# Autodesk Inventor assembly: 拨盘体
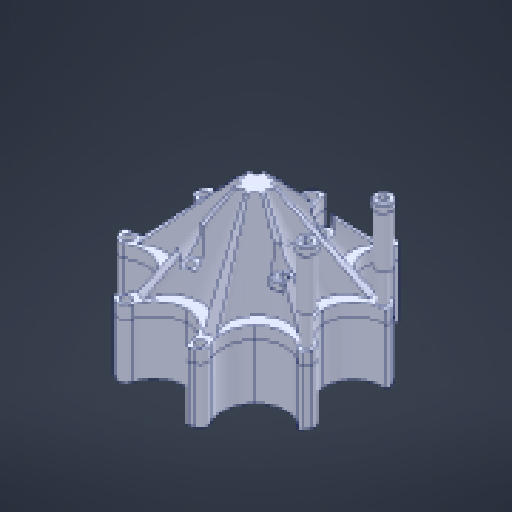
[picture p0: Inventor's stored thumbnail of the model, 512x512]
Saved by Autodesk Inventor 2025 (Build 290162000, 162)
## iProperties
Created: 2025-12-23
Part Number: 拨盘体
Document SubType Name: Assembly
Designer: XH
Author: XH
Revision Number: ä»
## Documents named in this file (8)
- C:\1A_Engineering_files\RCInventor\铝件版本\拨弹盘\拨盘体.iam
- C:\1A_Engineering_files\RCInventor\铝件版本\拨弹盘\八爪拨盘柱体.ipt
- C:\1A_Engineering_files\RCInventor\铝件版本\拨弹盘\八爪拨盘平面盘体.ipt
- C:\1A_Engineering_files\RCInventor\铝件版本\拨弹盘\2X铜嵌件M3-外5-长8.ipt
- C:\1A_Engineering_files\RCInventor\铝件版本\拨弹盘\螺栓M3-30.ipt
- C:\1A_Engineering_files\RCInventor\铝件版本\拨弹盘\斜坡滑槽.ipt
- C:\1A_Engineering_files\RCInventor\铝件版本\拨弹盘\螺栓M3-10.ipt
- C:\1A_Engineering_files\RCInventor\铝件版本\拨弹盘\螺栓M3-12.ipt
## Components (10 placed, 10 different names)
1. 八爪拨盘柱体_11 — 配合:1, 配合:2, 配合:3
2. 八爪拨盘平面盘体_12 — 配合:1, 配合:2, 配合:3
3. 螺栓M3-30_18
4. 螺栓M3-30_19
5. 2X铜嵌件M3-外5-长8_25
6. 2X铜嵌件M3-外5-长8_26
7. 斜坡滑槽_29
8. 螺栓M3-10_31
9. 螺栓M3-12_34
10. 螺栓M3-12_35
## Relationships (3: Mate 3)
- 配合:1 [Mate]: 八爪拨盘柱体_11 ↔ 八爪拨盘平面盘体_12
- 配合:2 [Mate]: 八爪拨盘柱体_11 ↔ 八爪拨盘平面盘体_12
- 配合:3 [Mate]: 八爪拨盘柱体_11 ↔ 八爪拨盘平面盘体_12
